# Autodesk Inventor assembly: Holder
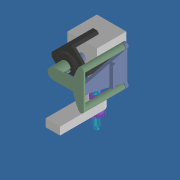
[picture p0: Inventor's stored thumbnail of the model, 180x180]
Saved by Autodesk Inventor 2020 (Build 240168000, 168)
## iProperties
Created: 2019-12-14
Part Number: Holder
Document SubType Name: Assembly
Designer: Jack
Author: Jack
## Documents named in this file (8)
- D:\SIT\EV3\Holder.iam
- D:\SIT\EV3\HolderGear.ipt
- D:\SIT\EV3\HolderShaft.ipt
- D:\SIT\EV3\Cube Cage.ipt
- D:\SIT\EV3\Cube.ipt
- D:\SIT\EV3\Hand.ipt
- D:\SIT\EV3\HandGear.ipt
- D:\SIT\EV3\HandSupport.ipt
## Components (7 placed, 7 different names)
1. HolderShaft:1 — Flush:1, Mate:2, Mate:3, Flush:2
2. HolderGear:1 — Flush:1, Mate:4, Angle:1, Angle:2, Mate:7, Mate:11
3. Cube Cage:1 — Mate:2, Mate:3, Mate:4, Mate:5, Mate:6, Mate:7, Angle:3
4. Cube:1 — Mate:5, Angle:1, Angle:2, Mate:6, Angle:3
5. Hand:1 — Cylindrical:1
6. HandGear:1 — Mate:11, Cylindrical:1, Mate:12
7. HandSupport:1 — Mate:12, Flush:2
## Relationships (14: Mate 8, Angle 3, Flush 2, CylindricalJoint 1)
- Flush:1: HolderShaft:1 ↔ HolderGear:1
- Mate:2: HolderShaft:1 ↔ Cube Cage:1
- Mate:3: HolderShaft:1 ↔ Cube Cage:1
- Mate:4: HolderGear:1 ↔ Cube Cage:1
- Mate:5: Cube Cage:1 ↔ Cube:1
- Angle:1 (0 deg): HolderGear:1 ↔ Cube:1
- Angle:2 (0 deg): HolderGear:1 ↔ Cube:1
- Mate:6: Cube Cage:1 ↔ Cube:1
- Mate:7 (12 mm): HolderGear:1 ↔ Cube Cage:1
- Angle:3 (0 deg): Cube Cage:1 ↔ Cube:1
- Mate:11 (40 mm): HolderGear:1 ↔ HandGear:1
- Cylindrical:1: Hand:1 ↔ HandGear:1
- Mate:12: HandGear:1 ↔ HandSupport:1
- Flush:2: HolderShaft:1 ↔ HandSupport:1
